# Autodesk Inventor assembly: wirePusher
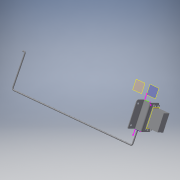
[picture p0: Inventor's stored thumbnail of the model, 180x180]
Saved by Autodesk Inventor 2017 (Build 210142000, 142)
## iProperties
Created: 2017-02-21
Part Number: wirePusher
Document SubType Name: Assembly
Designer: kingb
Author: kingb
## Documents named in this file (4)
- C:\Users\admin\Desktop\CAD\wirePusher.iam
- C:\Users\admin\Desktop\CAD\wirePusher.ipt
- C:\Users\admin\Desktop\CAD\HS-322HD.ipt
- C:\Users\admin\Desktop\CAD\HSmount.ipt
## Components (3 placed, 3 different names)
1. wirePusher:1 — Mate:1, Tangent:1
2. HS-322HD:1 — Mate:1, Tangent:1, Flush:1, Flush:2, Flush:3, Flush:4
3. HSmount:1 — Flush:2, Flush:3, Flush:4
## Relationships (6: Flush 4, Mate 1, Tangent 1)
- Mate:1: wirePusher:1 ↔ HS-322HD:1
- Tangent:1: wirePusher:1 ↔ HS-322HD:1
- Flush:1 (18.4912 mm): HS-322HD:1
- Flush:2: HS-322HD:1 ↔ HSmount:1
- Flush:3 (63.119 mm): HS-322HD:1 ↔ HSmount:1
- Flush:4: HS-322HD:1 ↔ HSmount:1
